# Autodesk Inventor assembly: ASY HPR 200  Frame
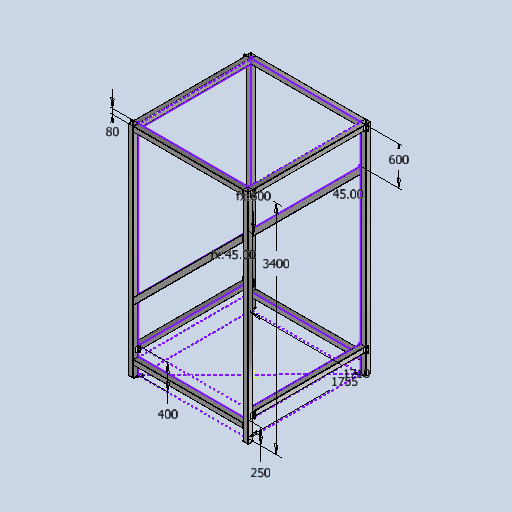
[picture p0: Inventor's stored thumbnail of the model, 512x512]
Saved by Autodesk Inventor 2025.1 (Build 291241020, 241B)
## iProperties
_SolveAssemblyDoc: Frame Generator Solve Assembly
_Version: 25.0.0
Created: 2024-11-03
Part Number: ASY HPR 200  Frame
Document SubType Name: Assembly
Designer: admin
Author: admin
## Documents named in this file (5)
- C:\Users\user\YandexDisk-badmisterfox\домашниий пк\Inventor\NDM-VOS_powder_hopper\ASY HPR 200  Frame.iam
- C:\Users\user\YandexDisk-badmisterfox\домашниий пк\Inventor\NDM-VOS_powder_hopper\NDM-VOS Рама Эскиз.ipt
- C:\Users\user\YandexDisk-badmisterfox\домашниий пк\Inventor\NDM-VOS_powder_hopper\ASY HPR 200  Frame\Frame\Frame 1730655523663.iam
- C:\Users\user\YandexDisk-badmisterfox\домашниий пк\Inventor\NDM-VOS_powder_hopper\NDM-VOS 912 flange slipway.ipt
- C:\Users\user\YandexDisk-badmisterfox\домашниий пк\Inventor\NDM-VOS_powder_hopper\NDM-VOS 901 base plate.ipt
## Components (30 placed, 4 different names)
1. NDM-VOS Рама Эскиз:1 — Mate:1, Flush:5, Flush:4
2. Frame 1730655523663:1 [sub-assembly] — Rigid:1, Rigid:3, Rigid:7, Rigid:8, Rigid:9, Rigid:16, Rigid:17, Rigid:18, Rigid:19, Rigid:20, Rigid:21, Rigid:24, Rigid:25, Rigid:26, Rigid:27, Rigid:28
3. NDM-VOS 912 flange slipway:1 — Rigid:2, Rigid:3
4. NDM-VOS 901 base plate:1 — Rigid:1
5. NDM-VOS 912 flange slipway:2 — Rigid:2
6. NDM-VOS 912 flange slipway:3 — Rigid:9
7. NDM-VOS 912 flange slipway:4
8. NDM-VOS 912 flange slipway:5 — Rigid:8
9. NDM-VOS 912 flange slipway:6
10. NDM-VOS 912 flange slipway:7 — Rigid:7
11. NDM-VOS 912 flange slipway:8
12. NDM-VOS 912 flange slipway:9 — Rigid:17
13. NDM-VOS 912 flange slipway:10
14. NDM-VOS 912 flange slipway:11
15. NDM-VOS 912 flange slipway:12 — Rigid:16
16. NDM-VOS 912 flange slipway:13
17. NDM-VOS 912 flange slipway:14 — Rigid:20
18. NDM-VOS 912 flange slipway:15 — Rigid:19
19. NDM-VOS 912 flange slipway:16
20. NDM-VOS 912 flange slipway:17
21. NDM-VOS 912 flange slipway:18 — Rigid:21
22. NDM-VOS 912 flange slipway:19 — Rigid:18
23. NDM-VOS 912 flange slipway:20
24. NDM-VOS 912 flange slipway:21
25. NDM-VOS 912 flange slipway:22 — Rigid:24
26. NDM-VOS 912 flange slipway:23
27. NDM-VOS 912 flange slipway:24 — Rigid:25
28. NDM-VOS 901 base plate:2 — Rigid:28
29. NDM-VOS 901 base plate:3 — Rigid:27
30. NDM-VOS 901 base plate:4 — Rigid:26
## Relationships (31: WeldJoint 28, Flush 2, Mate 1)
- Mate:1: NDM-VOS Рама Эскиз:1
- Flush:5: NDM-VOS Рама Эскиз:1
- Flush:4: NDM-VOS Рама Эскиз:1
- Rigid:1 [WeldJoint]: Frame 1730655523663:1 ↔ NDM-VOS 901 base plate:1
- Rigid:2 [WeldJoint]: NDM-VOS 912 flange slipway:1 ↔ NDM-VOS 912 flange slipway:2
- Rigid:3 [WeldJoint]: Frame 1730655523663:1 ↔ NDM-VOS 912 flange slipway:1
- [WeldJoint]: NDM-VOS 912 flange slipway:3 ↔ NDM-VOS 912 flange slipway:4
- [WeldJoint]: NDM-VOS 912 flange slipway:5 ↔ NDM-VOS 912 flange slipway:6
- [WeldJoint]: NDM-VOS 912 flange slipway:7 ↔ NDM-VOS 912 flange slipway:8
- Rigid:7 [WeldJoint]: Frame 1730655523663:1 ↔ NDM-VOS 912 flange slipway:7
- Rigid:8 [WeldJoint]: Frame 1730655523663:1 ↔ NDM-VOS 912 flange slipway:5
- Rigid:9 [WeldJoint]: Frame 1730655523663:1 ↔ NDM-VOS 912 flange slipway:3
- [WeldJoint]: NDM-VOS 912 flange slipway:9 ↔ NDM-VOS 912 flange slipway:10
- [WeldJoint]: NDM-VOS 912 flange slipway:11 ↔ NDM-VOS 912 flange slipway:12
- [WeldJoint]: NDM-VOS 912 flange slipway:13 ↔ NDM-VOS 912 flange slipway:14
- [WeldJoint]: NDM-VOS 912 flange slipway:15 ↔ NDM-VOS 912 flange slipway:16
- [WeldJoint]: NDM-VOS 912 flange slipway:17 ↔ NDM-VOS 912 flange slipway:18
- [WeldJoint]: NDM-VOS 912 flange slipway:19 ↔ NDM-VOS 912 flange slipway:20
- Rigid:16 [WeldJoint]: Frame 1730655523663:1 ↔ NDM-VOS 912 flange slipway:12
- Rigid:17 [WeldJoint]: Frame 1730655523663:1 ↔ NDM-VOS 912 flange slipway:9
- Rigid:18 [WeldJoint]: Frame 1730655523663:1 ↔ NDM-VOS 912 flange slipway:19
- Rigid:19 [WeldJoint]: Frame 1730655523663:1 ↔ NDM-VOS 912 flange slipway:15
- Rigid:20 [WeldJoint]: Frame 1730655523663:1 ↔ NDM-VOS 912 flange slipway:14
- Rigid:21 [WeldJoint]: Frame 1730655523663:1 ↔ NDM-VOS 912 flange slipway:18
- [WeldJoint]: NDM-VOS 912 flange slipway:21 ↔ NDM-VOS 912 flange slipway:22
- [WeldJoint]: NDM-VOS 912 flange slipway:23 ↔ NDM-VOS 912 flange slipway:24
- Rigid:24 [WeldJoint]: Frame 1730655523663:1 ↔ NDM-VOS 912 flange slipway:22
- Rigid:25 [WeldJoint]: Frame 1730655523663:1 ↔ NDM-VOS 912 flange slipway:24
- Rigid:26 [WeldJoint]: Frame 1730655523663:1 ↔ NDM-VOS 901 base plate:4
- Rigid:27 [WeldJoint]: Frame 1730655523663:1 ↔ NDM-VOS 901 base plate:3
- Rigid:28 [WeldJoint]: Frame 1730655523663:1 ↔ NDM-VOS 901 base plate:2
## Named parameters: d7_d5 = 0 mm, d8_d5 = 0 mm, d9_d5 = 0 mm, d13_d8_d5 = 0 mm, d14_d8_d5 = 0 mm, d15_d8_d5 = 0 mm, d16_d8_d5 = 0 mm, d17_d8_d5 = 0 mm, d18_d8_d5 = 0 mm, d25_d8_d5 = 0 mm, d26_d8_d5 = 0 mm
